# Autodesk Inventor assembly: søjle
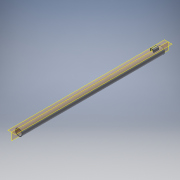
[picture p0: Inventor's stored thumbnail of the model, 180x180]
Saved by Autodesk Inventor 2018 (Build 220112000, 112)
## iProperties
Created: 2019-09-25
Part Number: søjle
Document SubType Name: Assembly
Designer: loppen
Author: loppen
## Documents named in this file (3)
- Z:\trappe\søjle\søjle.iam
- Z:\trappe\søjle\rør.ipt
- Z:\trappe\søjle\øre.ipt
## Components (2 placed, 2 different names)
1. rør:1 — Mate:1, Tangent:1
2. øre:1 — Mate:1, Tangent:1
## Relationships (2: Mate 1, Tangent 1)
- Mate:1: rør:1 ↔ øre:1
- Tangent:1: rør:1 ↔ øre:1
